# Autodesk Inventor assembly: Ensamble electroválvula y bobina
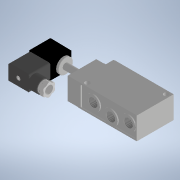
[picture p0: Inventor's stored thumbnail of the model, 180x180]
Saved by Autodesk Inventor 2021 (Build 250183000, 183)
## iProperties
Created: 2021-05-25
Part Number: Ensamble electroválvula y bobina
Document SubType Name: Assembly
Designer: Nelson
Mass: 345 g
Surface Area: 373.367 cm^2
Volume: 169.098 cm^3
Density: 2.04023 g/cm^3
Author: Nelson
## Documents named in this file (3)
- D:\Nelson\Documentos\Inventor\Proyecto_PAI\Ensamble electroválvula y bobina.iam
- D:\Nelson\Documentos\Inventor\Proyecto_PAI\Electrovalvula-5_2.ipt
- D:\Nelson\Documentos\Inventor\Proyecto_PAI\Bobina_Electrovalvula.iam
## Components (2 placed, 2 different names)
1. Electrovalvula-5_2:1 — Mate:1, Mate:2
2. Bobina_Electrovalvula:1 [sub-assembly] — Mate:1, Mate:2
## Relationships (2: Mate 2)
- Mate:1: Electrovalvula-5_2:1 ↔ Bobina_Electrovalvula:1
- Mate:2 (-6.406 mm): Electrovalvula-5_2:1 ↔ Bobina_Electrovalvula:1
